# Autodesk Inventor assembly: leftBackWing
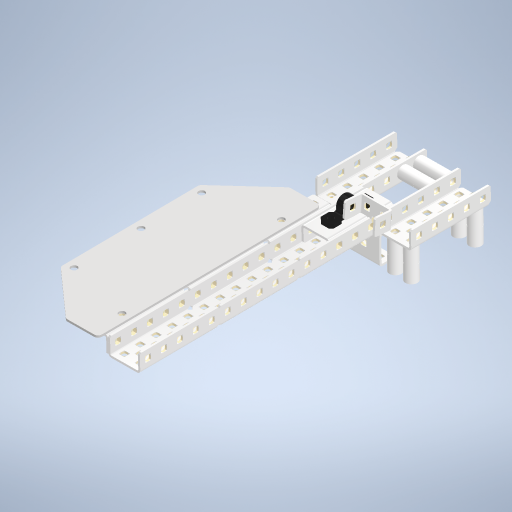
[picture p0: Inventor's stored thumbnail of the model, 512x512]
Saved by Autodesk Inventor 2023.4 (Build 274418000, 418)
## iProperties
Created: 2023-12-19
Part Number: leftBackWing
Document SubType Name: Assembly
Designer: Meer
Author: Meer
## Documents named in this file (10)
- C:\Users\Meer\OneDrive\Documents\GitHub\2024-599Z\Cad\leftBackWing.iam
- C:\Users\Meer\OneDrive\Documents\GitHub\2024-599Z\Cad\Library\VEX-CAD-Inventor-1.4.0\Structure\Gussets\C Channel Coupler.ipt
- C:\Users\Meer\OneDrive\Documents\GitHub\2024-599Z\Cad\Library\VEX-CAD-Inventor-1.4.0\Structure\C Channel\Aluminum 1x2x1\Alu C 1x2x1x16.ipt
- C:\Users\Meer\OneDrive\Documents\GitHub\2024-599Z\Cad\Library\VEX-CAD-Inventor-1.4.0\Motion\Shaft LS\LS Pillow Bearing Block.ipt
- C:\Users\Meer\OneDrive\Documents\GitHub\2024-599Z\Cad\Library\VEX-CAD-Inventor-1.4.0\Structure\C Channel\Aluminum 1x2x1\Alu C 1x2x1x5.ipt
- C:\Users\Meer\OneDrive\Documents\GitHub\2024-599Z\Cad\Library\VEX-CAD-Inventor-1.4.0\Motion\Spacers\Spacer Nylon .313 OD\NSpacer .313 OD x .500.ipt
- C:\Users\Meer\OneDrive\Documents\GitHub\2024-599Z\Cad\Library\VEX-CAD-Inventor-1.4.0\Motion\Spacers\Spacer Nylon .313 OD.ipt
- C:\Users\Meer\OneDrive\Documents\GitHub\2024-599Z\Cad\Library\VEX-CAD-Inventor-1.4.0\Structure\C Channel\Aluminum 1x2x1\Alu C 1x2x1x1.ipt
- C:\Users\Meer\OneDrive\Documents\GitHub\2024-599Z\Cad\NEW CNC Poly\wedge.ipt
- C:\Users\Meer\OneDrive\Documents\GitHub\2024-599Z\Cad\Library\VEX-CAD-Inventor-1.4.0\Structure\C Channel\Aluminum 1x3x1 Half\Alu C Half 1x3x1x14.ipt
## Components (21 placed, 8 different names)
1. C Channel Coupler:1
2. Alu C 1x2x1x16:1
3. LS Pillow Bearing Block:1
4. Alu C 1x2x1x5:1
5. NSpacer .313 OD x .500:1
6. NSpacer .313 OD x .500:2
7. NSpacer .313 OD x .500:3
8. NSpacer .313 OD x .500:4
9. Alu C 1x2x1x5:2
10. NSpacer .313 OD x .500:5
11. NSpacer .313 OD x .500:6
12. NSpacer .313 OD x .500:7
13. NSpacer .313 OD x .500:8
14. NSpacer .313 OD x .500:9
15. NSpacer .313 OD x .500:10
16. NSpacer .313 OD x .500:11
17. NSpacer .313 OD x .500:12
18. Alu C 1x2x1x1:1
19. C Channel Coupler:2
20. wedge:1
21. Alu C Half 1x3x1x14:1
## Relationships (24: Insert 23, Mate 1)
- [Mate]: C Channel Coupler:1 ↔ Alu C 1x2x1x16:1
- [Insert]: C Channel Coupler:1 ↔ LS Pillow Bearing Block:1
- [Insert]: Alu C 1x2x1x16:1 ↔ Alu C 1x2x1x5:1
- [Insert]: NSpacer .313 OD x .500:1 ↔ NSpacer .313 OD x .500:2
- [Insert]: NSpacer .313 OD x .500:3 ↔ NSpacer .313 OD x .500:4
- [Insert]: NSpacer .313 OD x .500:1 ↔ Alu C 1x2x1x5:2
- [Insert]: NSpacer .313 OD x .500:3 ↔ Alu C 1x2x1x5:2
- [Insert]: NSpacer .313 OD x .500:5 ↔ NSpacer .313 OD x .500:6
- [Insert]: Alu C 1x2x1x5:2 ↔ NSpacer .313 OD x .500:5
- [Insert]: NSpacer .313 OD x .500:7 ↔ NSpacer .313 OD x .500:8
- [Insert]: Alu C 1x2x1x5:2 ↔ NSpacer .313 OD x .500:8
- [Insert]: Alu C 1x2x1x5:2 ↔ NSpacer .313 OD x .500:5
- [Insert]: NSpacer .313 OD x .500:11 ↔ NSpacer .313 OD x .500:12
- [Insert]: Alu C 1x2x1x5:1 ↔ NSpacer .313 OD x .500:12
- [Insert]: Alu C 1x2x1x5:2 ↔ NSpacer .313 OD x .500:11
- [Insert]: NSpacer .313 OD x .500:9 ↔ NSpacer .313 OD x .500:10
- [Insert]: Alu C 1x2x1x5:1 ↔ NSpacer .313 OD x .500:10
- [Insert]: Alu C 1x2x1x5:2 ↔ NSpacer .313 OD x .500:9
- [Insert]: C Channel Coupler:1 ↔ Alu C 1x2x1x16:1
- [Insert]: LS Pillow Bearing Block:1 ↔ Alu C 1x2x1x1:1
- [Insert]: Alu C 1x2x1x16:1 ↔ Alu C Half 1x3x1x14:1
- [Insert]: Alu C 1x2x1x16:1 ↔ Alu C Half 1x3x1x14:1
- [Insert]: wedge:1 ↔ Alu C Half 1x3x1x14:1
- [Insert]: wedge:1 ↔ Alu C Half 1x3x1x14:1
## Named parameters: d1349_d1345 = 0 mm, d1351_d1345 = 0 mm
